# Autodesk Inventor assembly: ProvedoSenzor
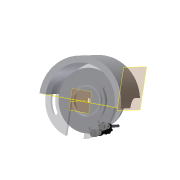
[picture p0: Inventor's stored thumbnail of the model, 180x180]
Saved by Autodesk Inventor 2015 SP1 (Build 190203100, 203)
## iProperties
Created: 2014-11-14
Part Number: ProvedoSenzor
Document SubType Name: Assembly
Designer: laca
Author: laca
## Documents named in this file (11)
- C:\Users\laca\Desktop\Allamvizsga\Invntor\RobotMechanikaForMAtlabVer2\ProvedoSenzor.iam
- C:\Users\laca\Desktop\Allamvizsga\Invntor\RobotMechanikaForMAtlabVer2\BurkolatPVCszenzor.ipt
- C:\Users\laca\Desktop\Allamvizsga\Invntor\RobotMechanikaForMAtlabVer2\PorvedoRogzitesAVazhoz.ipt
- C:\Users\laca\Desktop\Allamvizsga\Invntor\RobotMechanikaForMAtlabVer2\SzenzorSzuportKerek.ipt
- C:\Users\laca\Desktop\Allamvizsga\Invntor\RobotMechanikaForMAtlabVer2\InkrementalisOptikaiErzekelo.ipt
- C:\Users\laca\Desktop\Allamvizsga\Invntor\RobotMechanikaForMAtlabVer2\InkrementalisFolia.ipt
- C:\Users\laca\Desktop\Allamvizsga\Invntor\RobotMechanikaForMAtlabVer2\MerevitesInkrementalisFolia.ipt
- C:\Users\laca\Desktop\Allamvizsga\Invntor\RobotMechanikaForMAtlabVer2\Alatet3csavarhoz.ipt
- C:\Users\laca\Desktop\Allamvizsga\Invntor\RobotMechanikaForMAtlabVer2\Fi3es40mmcsavar Hexagon.ipt
- C:\Users\laca\Desktop\Allamvizsga\Invntor\RobotMechanikaForMAtlabVer2\3asAnya.ipt
- C:\Users\laca\Desktop\Allamvizsga\Invntor\RobotMechanikaForMAtlabVer2\KisLemezcsavar.ipt
## Components (21 placed, 10 different names)
1. PorvedoRogzitesAVazhoz:1 — Rotational:23, Insert:4, Flush:2, Rotational:28, Rotational:29, Rotational:32, Rotational:33
2. SzenzorSzuportKerek:1 — Rigid:1, Insert:2, Insert:3, Insert:4, Mate:1
3. InkrementalisFolia:1 — Insert:5, Flush:3
4. MerevitesInkrementalisFolia:1 — Rigid:1, Rigid:3
5. MerevitesInkrementalisFolia:2 — Rigid:3, Insert:5
6. KisLemezcsavar:1 — Insert:2
7. KisLemezcsavar:2 — Insert:3
8. BurkolatPVCszenzor:2 — Rotational:23, Flush:2
9. InkrementalisOptikaiErzekelo:2 — Cylindrical:1, Rotational:26, Rotational:27, Rotational:34, Rotational:35, Cylindrical:2, Flush:3
10. 3asAnya:5 — Rotational:27
11. 3asAnya:4 — Rotational:26
12. 3asAnya:2 — Rotational:25
13. Alatet3csavarhoz:6 — Rotational:25, Rotational:29
14. Alatet3csavarhoz:7 — Rotational:28
15. Fi3es40mmcsavar Hexagon:3 — Cylindrical:1
16. Alatet3csavarhoz:8 — Rotational:33
17. 3asAnya:6
18. Alatet3csavarhoz:9 — Rotational:32
19. Fi3es40mmcsavar Hexagon:4 — Cylindrical:2
20. 3asAnya:7 — Rotational:35
21. 3asAnya:8 — Rotational:34
## Relationships (24: RevoluteJoint 13, Insert 4, WeldJoint 2, CylindricalJoint 2, Flush 2, Mate 1)
- Rigid:1 [WeldJoint] (-8 mm): SzenzorSzuportKerek:1 ↔ MerevitesInkrementalisFolia:1
- [RevoluteJoint]: Alatet3csavarhoz:7 ↔ Fi3es40mmcsavar Hexagon:3
- Insert:2: SzenzorSzuportKerek:1 ↔ KisLemezcsavar:1
- Insert:3: SzenzorSzuportKerek:1 ↔ KisLemezcsavar:2
- Rigid:3 [WeldJoint]: MerevitesInkrementalisFolia:1 ↔ MerevitesInkrementalisFolia:2
- Rotational:23 [RevoluteJoint]: PorvedoRogzitesAVazhoz:1 ↔ BurkolatPVCszenzor:2
- Insert:4: PorvedoRogzitesAVazhoz:1 ↔ SzenzorSzuportKerek:1
- Rotational:25 [RevoluteJoint]: 3asAnya:2 ↔ Alatet3csavarhoz:6
- Cylindrical:1: InkrementalisOptikaiErzekelo:2 ↔ Fi3es40mmcsavar Hexagon:3
- Rotational:26 [RevoluteJoint]: InkrementalisOptikaiErzekelo:2 ↔ 3asAnya:4
- Rotational:27 [RevoluteJoint]: InkrementalisOptikaiErzekelo:2 ↔ 3asAnya:5
- Flush:2: PorvedoRogzitesAVazhoz:1 ↔ BurkolatPVCszenzor:2
- Mate:1: SzenzorSzuportKerek:1
- Rotational:28 [RevoluteJoint]: PorvedoRogzitesAVazhoz:1 ↔ Alatet3csavarhoz:7
- Rotational:29 [RevoluteJoint]: PorvedoRogzitesAVazhoz:1 ↔ Alatet3csavarhoz:6
- [RevoluteJoint]: Alatet3csavarhoz:9 ↔ Fi3es40mmcsavar Hexagon:4
- [RevoluteJoint]: Alatet3csavarhoz:8 ↔ 3asAnya:6
- Rotational:32 [RevoluteJoint]: PorvedoRogzitesAVazhoz:1 ↔ Alatet3csavarhoz:9
- Rotational:33 [RevoluteJoint]: PorvedoRogzitesAVazhoz:1 ↔ Alatet3csavarhoz:8
- Rotational:34 [RevoluteJoint]: InkrementalisOptikaiErzekelo:2 ↔ 3asAnya:8
- Rotational:35 [RevoluteJoint]: InkrementalisOptikaiErzekelo:2 ↔ 3asAnya:7
- Cylindrical:2: InkrementalisOptikaiErzekelo:2 ↔ Fi3es40mmcsavar Hexagon:4
- Insert:5: InkrementalisFolia:1 ↔ MerevitesInkrementalisFolia:2
- Flush:3 (2 mm): InkrementalisFolia:1 ↔ InkrementalisOptikaiErzekelo:2
## Named parameters: d72_d43 = 0 mm, d73_d46 = 4.867718 deg, d149_d123 = 0 mm, d150_d124 = 37.657506 deg, d151_d72_d43 = 0 mm, d152_d73_d46 = 140.861868 deg
